# Autodesk Inventor assembly: brush end effector
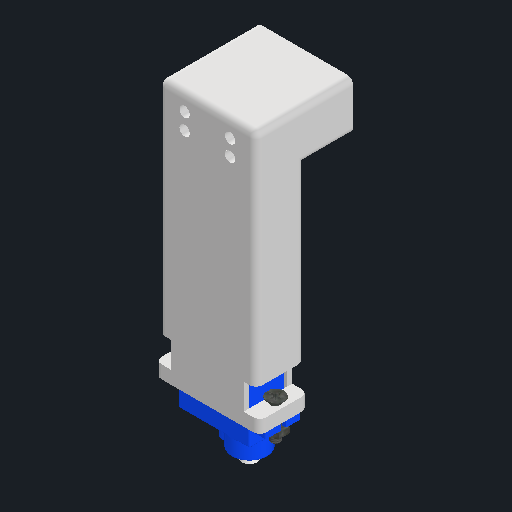
[picture p0: Inventor's stored thumbnail of the model, 512x512]
Saved by Autodesk Inventor 2024.2 (Build 282272000, 272)
## iProperties
Created: 2024-03-20
Part Number: brush end effector
Document SubType Name: Assembly
Designer: seifs
Author: seifs
## Documents named in this file (5)
- C:\Users\seifs\Downloads\Final Assembly\brush end effector.iam
- C:\Users\seifs\Downloads\Final Assembly\Servo Motor SG90.ipt
- C:\Users\seifs\Downloads\Final Assembly\attachment of brush.ipt
- C:\Users\seifs\OneDrive\Documents\Inventor\Content Center Files\R2024\en-US\ISO 7046-1 Z(1)\ISO 7046-1 - M3 x 12_ - 4.8 - Z - ISO.ipt
- C:\Users\seifs\OneDrive\Documents\Inventor\Content Center Files\R2024\en-US\ISO 4036(2)\ISO 4036 - M3(2).ipt
## Components (6 placed, 4 different names)
1. Servo Motor SG90:1 — Insert:1, Insert:2, Insert:16, Insert:17
2. attachment of brush:1 — Insert:1, Insert:2, Insert:14, Insert:15
3. ISO 7046-1 Z M3 x 12 - 4.8 - Z:2 — Insert:14
4. ISO 7046-1 Z M3 x 12 - 4.8 - Z:3 — Insert:15
5. ISO 4036 M3:2 — Insert:16
6. ISO 4036 M3:3 — Insert:17
## Relationships (6: Insert 6)
- Insert:1: Servo Motor SG90:1 ↔ attachment of brush:1
- Insert:2: Servo Motor SG90:1 ↔ attachment of brush:1
- Insert:14: attachment of brush:1 ↔ ISO 7046-1 Z M3 x 12 - 4.8 - Z:2
- Insert:15: attachment of brush:1 ↔ ISO 7046-1 Z M3 x 12 - 4.8 - Z:3
- Insert:16: Servo Motor SG90:1 ↔ ISO 4036 M3:2
- Insert:17: Servo Motor SG90:1 ↔ ISO 4036 M3:3
